# Autodesk Inventor assembly: 9P Sprocket
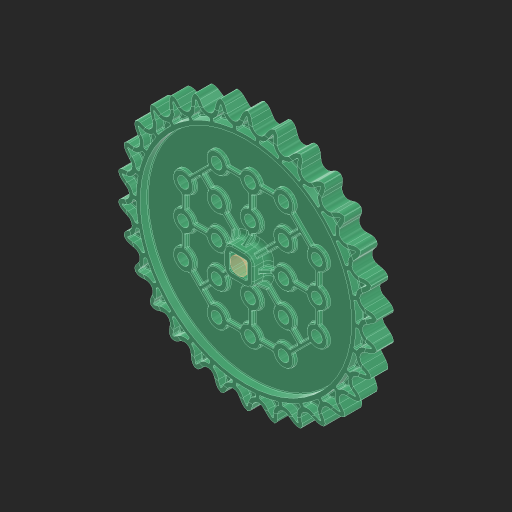
[picture p0: Inventor's stored thumbnail of the model, 512x512]
Saved by Autodesk Inventor 2023 (Build 270158000, 158)
## iProperties
Created: 2022-08-02
Part Number: 9P Sprocket
Document SubType Name: Assembly
Designer: ylu12
Author: ylu12
## Documents named in this file (3)
- C:\Users\ylu12\Documents\GitHub\VEX-CAD-Inventor\Motion\Sprockets\9P Sprocket\9P 30T Sprocket, No Insert.iam
- C:\Users\ylu12\Documents\GitHub\VEX-CAD-Inventor\Motion\Sprockets\Reference Files\9P 30T Sprocket, No Insert.ipt
- C:\Users\ylu12\Documents\GitHub\VEX-CAD-Inventor\Motion\Sprockets\9P Sprocket.iam
## Components (1 placed, 1 different names)
1. 30T — Mate:14, Mate:15, Mate:16
## Relationships (3: Mate 3)
- Mate:14: 30T
- Mate:15: 30T
- Mate:16: 30T
